# Autodesk Inventor assembly: New Updated Model
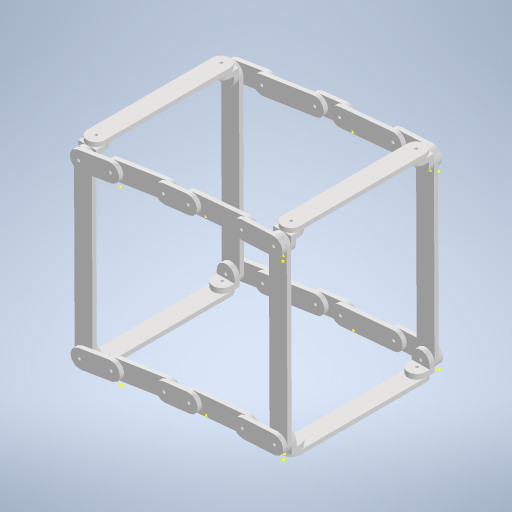
[picture p0: Inventor's stored thumbnail of the model, 512x512]
Saved by Autodesk Inventor 2024 (Build 280153000, 153)
## iProperties
Created: 2024-03-13
Part Number: New Updated Model
Document SubType Name: Assembly
Designer: ddcos
Author: ddcos
## Documents named in this file (7)
- C:\Users\ddcos\OneDrive\Documents\Project 4\Inventor\New Updated Model.iam
- C:\Users\ddcos\OneDrive\Documents\Project 4\Inventor\Vertical.ipt
- C:\Users\ddcos\OneDrive\Documents\Project 4\Inventor\Horizontal.ipt
- C:\Users\ddcos\OneDrive\Documents\Project 4\Inventor\Frame Connector.ipt
- C:\Users\ddcos\OneDrive\Documents\Project 4\Inventor\Small Rod.ipt
- C:\Users\ddcos\OneDrive\Documents\Project 4\Inventor\Middle.ipt
- C:\Users\ddcos\OneDrive\Documents\Project 4\Inventor\Large Rod.ipt
## Components (36 placed, 6 different names)
1. Vertical:1 — Mate:49, Mate:50, Mate:51, Mate:54, Mate:55
2. Vertical:2 — Mate:74, Mate:75, Mate:78, Mate:79
3. Horizontal:1
4. Horizontal:2
5. Frame Connector:1
6. Frame Connector:2
7. Frame Connector:3
8. Frame Connector:4
9. Vertical:3 — Mate:53, Mate:57
10. Vertical:4 — Mate:76, Mate:77, Mate:80, Mate:81
11. Horizontal:3
12. Horizontal:4
13. Frame Connector:5 — Mate:52
14. Frame Connector:6
15. Frame Connector:7
16. Frame Connector:8 — Mate:56
17. Small Rod:1 — Mate:33, Mate:34, Mate:54, Mate:55
18. Small Rod:2 — Mate:39, Mate:40, Mate:56, Mate:57
19. Small Rod:3 — Mate:58, Mate:59, Mate:78, Mate:79
20. Small Rod:4 — Mate:64, Mate:65, Mate:80, Mate:81
21. Middle:1 — Mate:35, Mate:36, Mate:37, Mate:38
22. Middle:2 — Mate:60, Mate:61, Mate:62, Mate:63
23. Large Rod:1 — Mate:33, Mate:34, Mate:35, Mate:36
24. Large Rod:2 — Mate:37, Mate:38, Mate:39, Mate:40
25. Large Rod:3 — Mate:62, Mate:63, Mate:64, Mate:65
26. Large Rod:4 — Mate:58, Mate:59, Mate:60, Mate:61
27. Small Rod:5 — Mate:49, Mate:50, Mate:51
28. Small Rod:6 — Mate:52, Mate:53
29. Middle:3
30. Large Rod:5
31. Large Rod:6
32. Small Rod:7 — Mate:74, Mate:75
33. Small Rod:8 — Mate:76, Mate:77
34. Middle:4
35. Large Rod:7
36. Large Rod:8
## Relationships (91: Mate 79, Flush 12)
- [Mate]: Vertical:1 ↔ Frame Connector:1
- [Mate]: Vertical:1 ↔ Frame Connector:1
- [Flush]: Vertical:1 ↔ Frame Connector:1
- [Mate]: Horizontal:1 ↔ Frame Connector:1
- [Mate]: Horizontal:1 ↔ Frame Connector:1
- [Flush]: Vertical:1 ↔ Horizontal:1
- [Mate]: Vertical:1 ↔ Frame Connector:4
- [Flush]: Vertical:1 ↔ Frame Connector:4
- [Mate]: Vertical:1 ↔ Frame Connector:4
- [Mate]: Horizontal:2 ↔ Frame Connector:4
- [Flush]: Vertical:1 ↔ Horizontal:2
- [Mate]: Horizontal:2 ↔ Frame Connector:4
- [Mate]: Horizontal:1 ↔ Frame Connector:2
- [Mate]: Horizontal:1 ↔ Frame Connector:2
- [Flush]: Horizontal:1 ↔ Frame Connector:2
- [Mate]: Horizontal:2 ↔ Frame Connector:3
- [Flush]: Horizontal:2 ↔ Frame Connector:3
- [Mate]: Horizontal:2 ↔ Frame Connector:3
- [Mate]: Vertical:2 ↔ Frame Connector:2
- [Mate]: Vertical:2 ↔ Frame Connector:3
- [Mate]: Vertical:2 ↔ Frame Connector:2
- [Mate]: Vertical:3 ↔ Frame Connector:5
- [Mate]: Vertical:3 ↔ Frame Connector:5
- [Flush]: Vertical:3 ↔ Frame Connector:5
- [Mate]: Horizontal:3 ↔ Frame Connector:5
- [Mate]: Horizontal:3 ↔ Frame Connector:5
- [Flush]: Vertical:3 ↔ Horizontal:3
- [Mate]: Vertical:3 ↔ Frame Connector:8
- [Flush]: Vertical:3 ↔ Frame Connector:8
- [Mate]: Vertical:3 ↔ Frame Connector:8
- [Mate]: Horizontal:4 ↔ Frame Connector:8
- [Flush]: Vertical:3 ↔ Horizontal:4
- [Mate]: Horizontal:4 ↔ Frame Connector:8
- [Mate]: Horizontal:3 ↔ Frame Connector:6
- [Mate]: Horizontal:3 ↔ Frame Connector:6
- [Flush]: Horizontal:3 ↔ Frame Connector:6
- [Mate]: Horizontal:4 ↔ Frame Connector:7
- [Flush]: Horizontal:4 ↔ Frame Connector:7
- [Mate]: Horizontal:4 ↔ Frame Connector:7
- [Mate]: Vertical:4 ↔ Frame Connector:6
- [Mate]: Vertical:4 ↔ Frame Connector:7
- [Mate]: Vertical:4 ↔ Frame Connector:6
- Mate:33: Small Rod:1 ↔ Large Rod:1
- Mate:34: Small Rod:1 ↔ Large Rod:1
- Mate:35: Middle:1 ↔ Large Rod:1
- Mate:36: Middle:1 ↔ Large Rod:1
- Mate:37: Middle:1 ↔ Large Rod:2
- Mate:38: Middle:1 ↔ Large Rod:2
- Mate:39: Small Rod:2 ↔ Large Rod:2
- Mate:40: Small Rod:2 ↔ Large Rod:2
- [Mate]: Small Rod:5 ↔ Large Rod:5
- [Mate]: Small Rod:5 ↔ Large Rod:5
- [Mate]: Middle:3 ↔ Large Rod:5
- [Mate]: Middle:3 ↔ Large Rod:5
- [Mate]: Middle:3 ↔ Large Rod:6
- [Mate]: Middle:3 ↔ Large Rod:6
- [Mate]: Small Rod:6 ↔ Large Rod:6
- [Mate]: Small Rod:6 ↔ Large Rod:6
- Mate:49: Vertical:1 ↔ Small Rod:5
- Mate:50: Vertical:1 ↔ Small Rod:5
- Mate:51: Vertical:1 ↔ Small Rod:5
- Mate:52: Frame Connector:5 ↔ Small Rod:6
- Mate:53: Vertical:3 ↔ Small Rod:6
- Mate:54: Vertical:1 ↔ Small Rod:1
- Mate:55: Vertical:1 ↔ Small Rod:1
- Mate:56: Frame Connector:8 ↔ Small Rod:2
- Mate:57: Vertical:3 ↔ Small Rod:2
- Mate:58: Small Rod:3 ↔ Large Rod:4
- Mate:59: Small Rod:3 ↔ Large Rod:4
- Mate:60: Middle:2 ↔ Large Rod:4
- Mate:61: Middle:2 ↔ Large Rod:4
- Mate:62: Middle:2 ↔ Large Rod:3
- Mate:63: Middle:2 ↔ Large Rod:3
- Mate:64: Small Rod:4 ↔ Large Rod:3
- Mate:65: Small Rod:4 ↔ Large Rod:3
- [Mate]: Small Rod:7 ↔ Large Rod:8
- [Mate]: Small Rod:7 ↔ Large Rod:8
- [Mate]: Middle:4 ↔ Large Rod:8
- [Mate]: Middle:4 ↔ Large Rod:8
- [Mate]: Middle:4 ↔ Large Rod:7
- [Mate]: Middle:4 ↔ Large Rod:7
- [Mate]: Small Rod:8 ↔ Large Rod:7
- [Mate]: Small Rod:8 ↔ Large Rod:7
- Mate:74: Vertical:2 ↔ Small Rod:7
- Mate:75: Vertical:2 ↔ Small Rod:7
- Mate:76: Vertical:4 ↔ Small Rod:8
- Mate:77: Vertical:4 ↔ Small Rod:8
- Mate:78: Vertical:2 ↔ Small Rod:3
- Mate:79: Vertical:2 ↔ Small Rod:3
- Mate:80: Vertical:4 ↔ Small Rod:4
- Mate:81: Vertical:4 ↔ Small Rod:4
## Named parameters: d21_d0 = 0 mm, d22_d12 = 0 mm, d23_d13 = 0 mm, d24_d14 = 0 mm, d25_d15 = 0 mm, d26_d16 = 0 mm, d27_d17 = 0 mm, d28_d18 = 0 mm, d29_d19 = 0 mm, d30_d20 = 0 mm, d31_d1 = 0 mm, d32_d2 = 0 mm, d33_d3 = 0 mm, d34_d4 = 0 mm, d35_d5 = 0 mm, d36_d6 = 0 mm, d37_d7 = 0 mm, d38_d8 = 0 mm, d39_d9 = 0 mm, d40_d10 = 0 mm, d41_d11 = 0 mm, d21_d21_d0 = 0 mm, d22_d22_d12 = 0 mm, d23_d23_d13 = 0 mm, d24_d24_d14 = 0 mm, d25_d25_d15 = 0 mm, d26_d26_d16 = 0 mm, d27_d27_d17 = 0 mm, d28_d28_d18 = 0 mm, d29_d29_d19 = 0 mm, d30_d30_d20 = 0 mm, d31_d31_d1 = 0 mm, d32_d32_d2 = 0 mm, d33_d33_d3 = 0 mm, d34_d34_d4 = 0 mm, d35_d35_d5 = 0 mm, d36_d36_d6 = 0 mm, d37_d37_d7 = 0 mm, d38_d38_d8 = 0 mm, d39_d39_d9 = 0 mm, d40_d40_d10 = 0 mm, d41_d41_d11 = 0 mm, d54_d47 = 0 mm, d55_d48 = 0 mm, d56_d49 = 0 mm, d57_d50 = 0 mm, d58_d51 = 0 mm, d59_d44 = 0 mm, d60_d45 = 0 mm, d61_d46 = 0 mm, d79_d71 = 0 mm, d80_d72 = 0 mm, d81_d73 = 0 mm, d82_d74 = 0 mm, d83_d75 = 0 mm, d84_d76 = 0 mm, d85_d77 = 0 mm, d86_d78 = 0 mm
